# Autodesk Inventor assembly: ballcaster
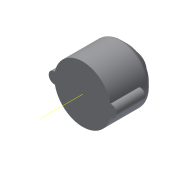
[picture p0: Inventor's stored thumbnail of the model, 180x180]
Saved by Autodesk Inventor 2014 (Build 180170000, 170)
## iProperties
Created: 2014-01-08
Part Number: ballcaster
Document SubType Name: Assembly
Designer: Felix
Author: Felix
## Documents named in this file (3)
- C:\Users\Felix\Desktop\Beep\Hardware\3D-CAD\ball_caster\ballcaster.iam
- C:\Users\Felix\Desktop\Beep\Hardware\3D-CAD\ball_caster\ball.ipt
- C:\Users\Felix\Desktop\Beep\Hardware\3D-CAD\ball_caster\case.ipt
## Components (2 placed, 2 different names)
1. ball:1 — Passend:1, Passend:2
2. case:1 — Passend:1, Passend:2
## Relationships (2: Mate 2)
- Passend:1 [Mate]: ball:1 ↔ case:1
- Passend:2 [Mate] (-10.2375 mm): ball:1 ↔ case:1
